# Autodesk Inventor assembly: Ball Bearing
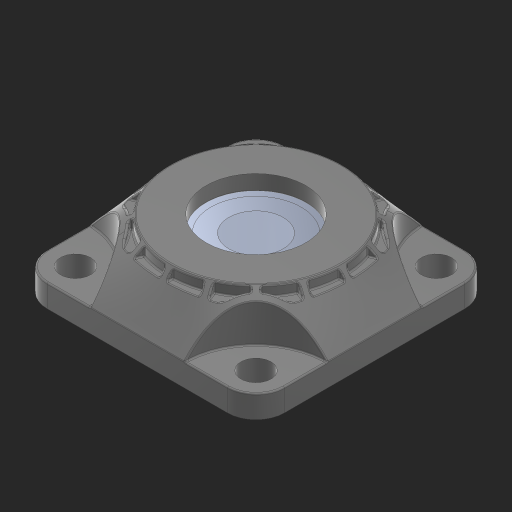
[picture p0: Inventor's stored thumbnail of the model, 512x512]
Saved by Autodesk Inventor 2023 (Build 270158000, 158)
## iProperties
Created: 2022-08-18
Part Number: Ball Bearing
Document SubType Name: Assembly
Designer: ylu12
Author: ylu12
## Documents named in this file (4)
- C:\Users\ylu12\Documents\GitHub\VEX-CAD-Inventor\Motion\Ball Bearing\Ball Bearing\Ball Bearing, No Insert.iam
- C:\Users\ylu12\Documents\GitHub\VEX-CAD-Inventor\Motion\Ball Bearing\Reference Files\Ball Bearing Housing.ipt
- C:\Users\ylu12\Documents\GitHub\VEX-CAD-Inventor\Motion\Ball Bearing\Reference Files\Ball Bearing.ipt
- C:\Users\ylu12\Documents\GitHub\VEX-CAD-Inventor\Motion\Ball Bearing\Ball Bearing.iam
## Components (2 placed, 2 different names)
1. Ball Bearing Housing:1 — Mate:1, Mate:2
2. Ball Bearing:1 — Mate:1, Mate:2
## Relationships (2: Mate 2)
- Mate:1: Ball Bearing Housing:1 ↔ Ball Bearing:1
- Mate:2: Ball Bearing Housing:1 ↔ Ball Bearing:1
